# Autodesk Inventor assembly: 7407-S1
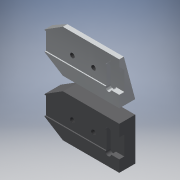
[picture p0: Inventor's stored thumbnail of the model, 180x180]
Saved by Autodesk Inventor 2018 (Build 220112000, 112)
## iProperties
Created: 2018-10-15
Part Number: 7407-S1
Project: =<Part Number>
Document SubType Name: Assembly
Designer: S.O.
Author: S.O.
## Documents named in this file (3)
- R:\CAD\~Aquafil~\7407 - 456 Slant Blades-72 Flat Blades (Standard Size)\CAD\7407-S1.iam
- R:\CAD\~Aquafil~\7407 - 456 Slant Blades-72 Flat Blades (Standard Size)\CAD\DHC-1500-FF-02-002.ipt
- R:\CAD\~Aquafil~\7407 - 456 Slant Blades-72 Flat Blades (Standard Size)\CAD\DHC-1500-FF-02-003.ipt
## Components (528 placed, 2 different names)
1. DHC-1500-FF-02-003:1 — Flush:1, Flush:2, Mate:1
2. DHC-1500-FF-02-003:2
3. DHC-1500-FF-02-003:3
4. DHC-1500-FF-02-003:4
5. DHC-1500-FF-02-003:5
6. DHC-1500-FF-02-003:6
7. DHC-1500-FF-02-003:7
8. DHC-1500-FF-02-003:8
9. DHC-1500-FF-02-003:9
10. DHC-1500-FF-02-003:10
11. DHC-1500-FF-02-003:11
12. DHC-1500-FF-02-003:12
13. DHC-1500-FF-02-003:13
14. DHC-1500-FF-02-003:14
15. DHC-1500-FF-02-003:15
16. DHC-1500-FF-02-003:16
17. DHC-1500-FF-02-003:17
18. DHC-1500-FF-02-003:18
19. DHC-1500-FF-02-003:19
20. DHC-1500-FF-02-003:20
21. DHC-1500-FF-02-003:21
22. DHC-1500-FF-02-003:22
23. DHC-1500-FF-02-003:23
24. DHC-1500-FF-02-003:24
25. DHC-1500-FF-02-003:25
26. DHC-1500-FF-02-003:26
27. DHC-1500-FF-02-003:27
28. DHC-1500-FF-02-003:28
29. DHC-1500-FF-02-003:29
30. DHC-1500-FF-02-003:30
31. DHC-1500-FF-02-003:31
32. DHC-1500-FF-02-003:32
33. DHC-1500-FF-02-003:33
34. DHC-1500-FF-02-003:34
35. DHC-1500-FF-02-003:35
36. DHC-1500-FF-02-003:36
37. DHC-1500-FF-02-003:37
38. DHC-1500-FF-02-003:38
39. DHC-1500-FF-02-003:39
40. DHC-1500-FF-02-003:40
41. DHC-1500-FF-02-003:41
42. DHC-1500-FF-02-003:42
43. DHC-1500-FF-02-003:43
44. DHC-1500-FF-02-003:44
45. DHC-1500-FF-02-003:45
46. DHC-1500-FF-02-003:46
47. DHC-1500-FF-02-003:47
48. DHC-1500-FF-02-003:48
49. DHC-1500-FF-02-003:49
50. DHC-1500-FF-02-003:50
51. DHC-1500-FF-02-003:51
52. DHC-1500-FF-02-003:52
53. DHC-1500-FF-02-003:53
54. DHC-1500-FF-02-003:54
55. DHC-1500-FF-02-003:55
56. DHC-1500-FF-02-003:56
57. DHC-1500-FF-02-003:57
58. DHC-1500-FF-02-003:58
59. DHC-1500-FF-02-003:59
60. DHC-1500-FF-02-003:60
61. DHC-1500-FF-02-003:61
62. DHC-1500-FF-02-003:62
63. DHC-1500-FF-02-003:63
64. DHC-1500-FF-02-003:64
65. DHC-1500-FF-02-003:65
66. DHC-1500-FF-02-003:66
67. DHC-1500-FF-02-003:67
68. DHC-1500-FF-02-003:68
69. DHC-1500-FF-02-003:69
70. DHC-1500-FF-02-003:70
71. DHC-1500-FF-02-003:71
72. DHC-1500-FF-02-003:72
73. DHC-1500-FF-02-003:73
74. DHC-1500-FF-02-003:74
75. DHC-1500-FF-02-003:75
76. DHC-1500-FF-02-003:76
77. DHC-1500-FF-02-003:77
78. DHC-1500-FF-02-003:78
79. DHC-1500-FF-02-003:79
80. DHC-1500-FF-02-003:80
81. DHC-1500-FF-02-003:81
82. DHC-1500-FF-02-003:82
83. DHC-1500-FF-02-003:83
84. DHC-1500-FF-02-003:84
85. DHC-1500-FF-02-003:85
86. DHC-1500-FF-02-003:86
87. DHC-1500-FF-02-003:87
88. DHC-1500-FF-02-003:88
89. DHC-1500-FF-02-003:89
90. DHC-1500-FF-02-003:90
91. DHC-1500-FF-02-003:91
92. DHC-1500-FF-02-003:92
93. DHC-1500-FF-02-003:93
94. DHC-1500-FF-02-003:94
95. DHC-1500-FF-02-003:95
96. DHC-1500-FF-02-003:96
97. DHC-1500-FF-02-003:97
98. DHC-1500-FF-02-003:98
99. DHC-1500-FF-02-003:99
100. DHC-1500-FF-02-003:100
101. DHC-1500-FF-02-003:101
102. DHC-1500-FF-02-003:102
103. DHC-1500-FF-02-003:103
104. DHC-1500-FF-02-003:104
105. DHC-1500-FF-02-003:105
106. DHC-1500-FF-02-003:106
107. DHC-1500-FF-02-003:107
108. DHC-1500-FF-02-003:108
109. DHC-1500-FF-02-003:109
110. DHC-1500-FF-02-003:110
111. DHC-1500-FF-02-003:111
112. DHC-1500-FF-02-003:112
113. DHC-1500-FF-02-003:113
114. DHC-1500-FF-02-003:114
115. DHC-1500-FF-02-003:115
116. DHC-1500-FF-02-003:116
117. DHC-1500-FF-02-003:117
118. DHC-1500-FF-02-003:118
119. DHC-1500-FF-02-003:119
120. DHC-1500-FF-02-003:120
121. DHC-1500-FF-02-003:121
122. DHC-1500-FF-02-003:122
123. DHC-1500-FF-02-003:123
124. DHC-1500-FF-02-003:124
125. DHC-1500-FF-02-003:125
126. DHC-1500-FF-02-003:126
127. DHC-1500-FF-02-003:127
128. DHC-1500-FF-02-003:128
129. DHC-1500-FF-02-003:129
130. DHC-1500-FF-02-003:130
131. DHC-1500-FF-02-003:131
132. DHC-1500-FF-02-003:132
133. DHC-1500-FF-02-003:133
134. DHC-1500-FF-02-003:134
135. DHC-1500-FF-02-003:135
136. DHC-1500-FF-02-003:136
137. DHC-1500-FF-02-003:137
138. DHC-1500-FF-02-003:138
139. DHC-1500-FF-02-003:139
140. DHC-1500-FF-02-003:140
141. DHC-1500-FF-02-003:141
142. DHC-1500-FF-02-003:142
143. DHC-1500-FF-02-003:143
144. DHC-1500-FF-02-003:144
145. DHC-1500-FF-02-003:145
146. DHC-1500-FF-02-003:146
147. DHC-1500-FF-02-003:147
148. DHC-1500-FF-02-003:148
149. DHC-1500-FF-02-003:149
150. DHC-1500-FF-02-003:150
151. DHC-1500-FF-02-003:151
152. DHC-1500-FF-02-003:152
153. DHC-1500-FF-02-003:153
154. DHC-1500-FF-02-003:154
155. DHC-1500-FF-02-003:155
156. DHC-1500-FF-02-003:156
157. DHC-1500-FF-02-003:157
158. DHC-1500-FF-02-003:158
159. DHC-1500-FF-02-003:159
160. DHC-1500-FF-02-003:160
161. DHC-1500-FF-02-003:161
162. DHC-1500-FF-02-003:162
163. DHC-1500-FF-02-003:163
164. DHC-1500-FF-02-003:164
165. DHC-1500-FF-02-003:165
166. DHC-1500-FF-02-003:166
167. DHC-1500-FF-02-003:167
168. DHC-1500-FF-02-003:168
169. DHC-1500-FF-02-003:169
170. DHC-1500-FF-02-003:170
171. DHC-1500-FF-02-003:171
172. DHC-1500-FF-02-003:172
173. DHC-1500-FF-02-003:173
174. DHC-1500-FF-02-003:174
175. DHC-1500-FF-02-003:175
176. DHC-1500-FF-02-003:176
177. DHC-1500-FF-02-003:177
178. DHC-1500-FF-02-003:178
179. DHC-1500-FF-02-003:179
180. DHC-1500-FF-02-003:180
181. DHC-1500-FF-02-003:181
182. DHC-1500-FF-02-003:182
183. DHC-1500-FF-02-003:183
184. DHC-1500-FF-02-003:184
185. DHC-1500-FF-02-003:185
186. DHC-1500-FF-02-003:186
187. DHC-1500-FF-02-003:187
188. DHC-1500-FF-02-003:188
189. DHC-1500-FF-02-003:189
190. DHC-1500-FF-02-003:190
191. DHC-1500-FF-02-003:191
192. DHC-1500-FF-02-003:192
193. DHC-1500-FF-02-003:193
194. DHC-1500-FF-02-003:194
195. DHC-1500-FF-02-003:195
196. DHC-1500-FF-02-003:196
197. DHC-1500-FF-02-003:197
198. DHC-1500-FF-02-003:198
199. DHC-1500-FF-02-003:199
200. DHC-1500-FF-02-003:200
201. DHC-1500-FF-02-003:201
202. DHC-1500-FF-02-003:202
203. DHC-1500-FF-02-003:203
204. DHC-1500-FF-02-003:204
205. DHC-1500-FF-02-003:205
206. DHC-1500-FF-02-003:206
207. DHC-1500-FF-02-003:207
208. DHC-1500-FF-02-003:208
209. DHC-1500-FF-02-003:209
210. DHC-1500-FF-02-003:210
211. DHC-1500-FF-02-003:211
212. DHC-1500-FF-02-003:212
213. DHC-1500-FF-02-003:213
214. DHC-1500-FF-02-003:214
215. DHC-1500-FF-02-003:215
216. DHC-1500-FF-02-003:216
217. DHC-1500-FF-02-003:217
218. DHC-1500-FF-02-003:218
219. DHC-1500-FF-02-003:219
220. DHC-1500-FF-02-003:220
221. DHC-1500-FF-02-003:221
222. DHC-1500-FF-02-003:222
223. DHC-1500-FF-02-003:223
224. DHC-1500-FF-02-003:224
225. DHC-1500-FF-02-003:225
226. DHC-1500-FF-02-003:226
227. DHC-1500-FF-02-003:227
228. DHC-1500-FF-02-003:228
229. DHC-1500-FF-02-003:229
230. DHC-1500-FF-02-003:230
231. DHC-1500-FF-02-003:231
232. DHC-1500-FF-02-003:232
233. DHC-1500-FF-02-003:233
234. DHC-1500-FF-02-003:234
235. DHC-1500-FF-02-003:235
236. DHC-1500-FF-02-003:236
237. DHC-1500-FF-02-003:237
238. DHC-1500-FF-02-003:238
239. DHC-1500-FF-02-003:239
240. DHC-1500-FF-02-003:240
241. DHC-1500-FF-02-003:241
242. DHC-1500-FF-02-003:242
243. DHC-1500-FF-02-003:243
244. DHC-1500-FF-02-003:244
245. DHC-1500-FF-02-003:245
246. DHC-1500-FF-02-003:246
247. DHC-1500-FF-02-003:247
248. DHC-1500-FF-02-003:248
249. DHC-1500-FF-02-003:249
250. DHC-1500-FF-02-003:250
251. DHC-1500-FF-02-003:251
252. DHC-1500-FF-02-003:252
253. DHC-1500-FF-02-003:253
254. DHC-1500-FF-02-003:254
255. DHC-1500-FF-02-003:255
256. DHC-1500-FF-02-003:256
257. DHC-1500-FF-02-003:257
258. DHC-1500-FF-02-003:258
259. DHC-1500-FF-02-003:259
260. DHC-1500-FF-02-003:260
261. DHC-1500-FF-02-003:261
262. DHC-1500-FF-02-003:262
263. DHC-1500-FF-02-003:263
264. DHC-1500-FF-02-003:264
265. DHC-1500-FF-02-003:265
266. DHC-1500-FF-02-003:266
267. DHC-1500-FF-02-003:267
268. DHC-1500-FF-02-003:268
269. DHC-1500-FF-02-003:269
270. DHC-1500-FF-02-003:270
271. DHC-1500-FF-02-003:271
272. DHC-1500-FF-02-003:272
273. DHC-1500-FF-02-003:273
274. DHC-1500-FF-02-003:274
275. DHC-1500-FF-02-003:275
276. DHC-1500-FF-02-003:276
277. DHC-1500-FF-02-003:277
278. DHC-1500-FF-02-003:278
279. DHC-1500-FF-02-003:279
280. DHC-1500-FF-02-003:280
281. DHC-1500-FF-02-003:281
282. DHC-1500-FF-02-003:282
283. DHC-1500-FF-02-003:283
284. DHC-1500-FF-02-003:284
285. DHC-1500-FF-02-003:285
286. DHC-1500-FF-02-003:286
287. DHC-1500-FF-02-003:287
288. DHC-1500-FF-02-003:288
289. DHC-1500-FF-02-003:289
290. DHC-1500-FF-02-003:290
291. DHC-1500-FF-02-003:291
292. DHC-1500-FF-02-003:292
293. DHC-1500-FF-02-003:293
294. DHC-1500-FF-02-003:294
295. DHC-1500-FF-02-003:295
296. DHC-1500-FF-02-003:296
297. DHC-1500-FF-02-003:297
298. DHC-1500-FF-02-003:298
299. DHC-1500-FF-02-003:299
300. DHC-1500-FF-02-003:300
301. DHC-1500-FF-02-003:301
302. DHC-1500-FF-02-003:302
303. DHC-1500-FF-02-003:303
304. DHC-1500-FF-02-003:304
305. DHC-1500-FF-02-003:305
306. DHC-1500-FF-02-003:306
307. DHC-1500-FF-02-003:307
308. DHC-1500-FF-02-003:308
309. DHC-1500-FF-02-003:309
310. DHC-1500-FF-02-003:310
311. DHC-1500-FF-02-003:311
312. DHC-1500-FF-02-003:312
313. DHC-1500-FF-02-003:313
314. DHC-1500-FF-02-003:314
315. DHC-1500-FF-02-003:315
316. DHC-1500-FF-02-003:316
317. DHC-1500-FF-02-003:317
318. DHC-1500-FF-02-003:318
319. DHC-1500-FF-02-003:319
320. DHC-1500-FF-02-003:320
321. DHC-1500-FF-02-003:321
322. DHC-1500-FF-02-003:322
323. DHC-1500-FF-02-003:323
324. DHC-1500-FF-02-003:324
325. DHC-1500-FF-02-003:325
326. DHC-1500-FF-02-003:326
327. DHC-1500-FF-02-003:327
328. DHC-1500-FF-02-003:328
329. DHC-1500-FF-02-003:329
330. DHC-1500-FF-02-003:330
331. DHC-1500-FF-02-003:331
332. DHC-1500-FF-02-003:332
333. DHC-1500-FF-02-003:333
334. DHC-1500-FF-02-003:334
335. DHC-1500-FF-02-003:335
336. DHC-1500-FF-02-003:336
337. DHC-1500-FF-02-003:337
338. DHC-1500-FF-02-003:338
339. DHC-1500-FF-02-003:339
340. DHC-1500-FF-02-003:340
341. DHC-1500-FF-02-003:341
342. DHC-1500-FF-02-003:342
343. DHC-1500-FF-02-003:343
344. DHC-1500-FF-02-003:344
345. DHC-1500-FF-02-003:345
346. DHC-1500-FF-02-003:346
347. DHC-1500-FF-02-003:347
348. DHC-1500-FF-02-003:348
349. DHC-1500-FF-02-003:349
350. DHC-1500-FF-02-003:350
351. DHC-1500-FF-02-003:351
352. DHC-1500-FF-02-003:352
353. DHC-1500-FF-02-003:353
354. DHC-1500-FF-02-003:354
355. DHC-1500-FF-02-003:355
356. DHC-1500-FF-02-003:356
357. DHC-1500-FF-02-003:357
358. DHC-1500-FF-02-003:358
359. DHC-1500-FF-02-003:359
360. DHC-1500-FF-02-003:360
361. DHC-1500-FF-02-003:361
362. DHC-1500-FF-02-003:362
363. DHC-1500-FF-02-003:363
364. DHC-1500-FF-02-003:364
365. DHC-1500-FF-02-003:365
366. DHC-1500-FF-02-003:366
367. DHC-1500-FF-02-003:367
368. DHC-1500-FF-02-003:368
369. DHC-1500-FF-02-003:369
370. DHC-1500-FF-02-003:370
371. DHC-1500-FF-02-003:371
372. DHC-1500-FF-02-003:372
373. DHC-1500-FF-02-003:373
374. DHC-1500-FF-02-003:374
375. DHC-1500-FF-02-003:375
376. DHC-1500-FF-02-003:376
377. DHC-1500-FF-02-003:377
378. DHC-1500-FF-02-003:378
379. DHC-1500-FF-02-003:379
380. DHC-1500-FF-02-003:380
381. DHC-1500-FF-02-003:381
382. DHC-1500-FF-02-003:382
383. DHC-1500-FF-02-003:383
384. DHC-1500-FF-02-003:384
385. DHC-1500-FF-02-003:385
386. DHC-1500-FF-02-003:386
387. DHC-1500-FF-02-003:387
388. DHC-1500-FF-02-003:388
389. DHC-1500-FF-02-003:389
390. DHC-1500-FF-02-003:390
391. DHC-1500-FF-02-003:391
392. DHC-1500-FF-02-003:392
393. DHC-1500-FF-02-003:393
394. DHC-1500-FF-02-003:394
395. DHC-1500-FF-02-003:395
396. DHC-1500-FF-02-003:396
397. DHC-1500-FF-02-003:397
398. DHC-1500-FF-02-003:398
399. DHC-1500-FF-02-003:399
400. DHC-1500-FF-02-003:400
401. DHC-1500-FF-02-003:401
402. DHC-1500-FF-02-003:402
403. DHC-1500-FF-02-003:403
404. DHC-1500-FF-02-003:404
405. DHC-1500-FF-02-003:405
406. DHC-1500-FF-02-003:406
407. DHC-1500-FF-02-003:407
408. DHC-1500-FF-02-003:408
409. DHC-1500-FF-02-003:409
410. DHC-1500-FF-02-003:410
411. DHC-1500-FF-02-003:411
412. DHC-1500-FF-02-003:412
413. DHC-1500-FF-02-003:413
414. DHC-1500-FF-02-003:414
415. DHC-1500-FF-02-003:415
416. DHC-1500-FF-02-003:416
417. DHC-1500-FF-02-003:417
418. DHC-1500-FF-02-003:418
419. DHC-1500-FF-02-003:419
420. DHC-1500-FF-02-003:420
421. DHC-1500-FF-02-003:421
422. DHC-1500-FF-02-003:422
423. DHC-1500-FF-02-003:423
424. DHC-1500-FF-02-003:424
425. DHC-1500-FF-02-003:425
426. DHC-1500-FF-02-003:426
427. DHC-1500-FF-02-003:427
428. DHC-1500-FF-02-003:428
429. DHC-1500-FF-02-003:429
430. DHC-1500-FF-02-003:430
431. DHC-1500-FF-02-003:431
432. DHC-1500-FF-02-003:432
433. DHC-1500-FF-02-003:433
434. DHC-1500-FF-02-003:434
435. DHC-1500-FF-02-003:435
436. DHC-1500-FF-02-003:436
437. DHC-1500-FF-02-003:437
438. DHC-1500-FF-02-003:438
439. DHC-1500-FF-02-003:439
440. DHC-1500-FF-02-003:440
441. DHC-1500-FF-02-003:441
442. DHC-1500-FF-02-003:442
443. DHC-1500-FF-02-003:443
444. DHC-1500-FF-02-003:444
445. DHC-1500-FF-02-003:445
446. DHC-1500-FF-02-003:446
447. DHC-1500-FF-02-003:447
448. DHC-1500-FF-02-003:448
449. DHC-1500-FF-02-003:449
450. DHC-1500-FF-02-003:450
451. DHC-1500-FF-02-003:451
452. DHC-1500-FF-02-003:452
453. DHC-1500-FF-02-003:453
454. DHC-1500-FF-02-003:454
455. DHC-1500-FF-02-003:455
456. DHC-1500-FF-02-003:456
457. DHC-1500-FF-02-002:1 — Flush:1, Flush:2, Mate:1
458. DHC-1500-FF-02-002:2
459. DHC-1500-FF-02-002:3
460. DHC-1500-FF-02-002:4
461. DHC-1500-FF-02-002:5
462. DHC-1500-FF-02-002:6
463. DHC-1500-FF-02-002:7
464. DHC-1500-FF-02-002:8
465. DHC-1500-FF-02-002:9
466. DHC-1500-FF-02-002:10
467. DHC-1500-FF-02-002:11
468. DHC-1500-FF-02-002:12
469. DHC-1500-FF-02-002:13
470. DHC-1500-FF-02-002:14
471. DHC-1500-FF-02-002:15
472. DHC-1500-FF-02-002:16
473. DHC-1500-FF-02-002:17
474. DHC-1500-FF-02-002:18
475. DHC-1500-FF-02-002:19
476. DHC-1500-FF-02-002:20
477. DHC-1500-FF-02-002:21
478. DHC-1500-FF-02-002:22
479. DHC-1500-FF-02-002:23
480. DHC-1500-FF-02-002:24
481. DHC-1500-FF-02-002:25
482. DHC-1500-FF-02-002:26
483. DHC-1500-FF-02-002:27
484. DHC-1500-FF-02-002:28
485. DHC-1500-FF-02-002:29
486. DHC-1500-FF-02-002:30
487. DHC-1500-FF-02-002:31
488. DHC-1500-FF-02-002:32
489. DHC-1500-FF-02-002:33
490. DHC-1500-FF-02-002:34
491. DHC-1500-FF-02-002:35
492. DHC-1500-FF-02-002:36
493. DHC-1500-FF-02-002:37
494. DHC-1500-FF-02-002:38
495. DHC-1500-FF-02-002:39
496. DHC-1500-FF-02-002:40
497. DHC-1500-FF-02-002:41
498. DHC-1500-FF-02-002:42
499. DHC-1500-FF-02-002:43
500. DHC-1500-FF-02-002:44
501. DHC-1500-FF-02-002:45
502. DHC-1500-FF-02-002:46
503. DHC-1500-FF-02-002:47
504. DHC-1500-FF-02-002:48
505. DHC-1500-FF-02-002:49
506. DHC-1500-FF-02-002:50
507. DHC-1500-FF-02-002:51
508. DHC-1500-FF-02-002:52
509. DHC-1500-FF-02-002:53
510. DHC-1500-FF-02-002:54
511. DHC-1500-FF-02-002:55
512. DHC-1500-FF-02-002:56
513. DHC-1500-FF-02-002:57
514. DHC-1500-FF-02-002:58
515. DHC-1500-FF-02-002:59
516. DHC-1500-FF-02-002:60
517. DHC-1500-FF-02-002:61
518. DHC-1500-FF-02-002:62
519. DHC-1500-FF-02-002:63
520. DHC-1500-FF-02-002:64
521. DHC-1500-FF-02-002:65
522. DHC-1500-FF-02-002:66
523. DHC-1500-FF-02-002:67
524. DHC-1500-FF-02-002:68
525. DHC-1500-FF-02-002:69
526. DHC-1500-FF-02-002:70
527. DHC-1500-FF-02-002:71
528. DHC-1500-FF-02-002:72
## Component patterns: (456 elements, first: DHC-1500-FF-02-003:1), (72 elements, first: DHC-1500-FF-02-002:1)
## Relationships (3: Flush 2, Mate 1)
- Flush:1: DHC-1500-FF-02-003:1 ↔ DHC-1500-FF-02-002:1
- Flush:2: DHC-1500-FF-02-003:1 ↔ DHC-1500-FF-02-002:1
- Mate:1 (25.4 mm): DHC-1500-FF-02-003:1 ↔ DHC-1500-FF-02-002:1
